# Autodesk Inventor assembly: ForeArm
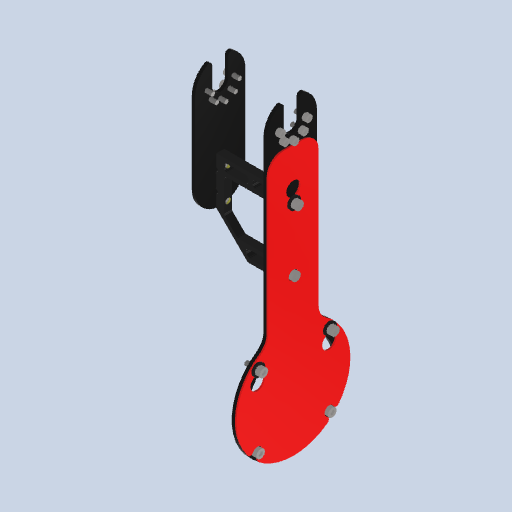
[picture p0: Inventor's stored thumbnail of the model, 512x512]
Saved by Autodesk Inventor 2022.3 (Build 263350000, 350)
## iProperties
Created: 2022-01-11
Part Number: ForeArm
Document SubType Name: Assembly
Designer: Masato Kubotera
Author: Masato Kubotera
## Documents named in this file (10)
- C:\Users\Masato\Documents\Inventor\CIT Brains\SUSTAINA-OP - mod\UpperBody\Arm\ForeArm.iam
- C:\Users\Masato\Documents\Inventor\CIT Brains\SUSTAINA-OP - mod\UpperBody\Arm\ForeArm_outside_frame.ipt
- C:\Users\Masato\Documents\Inventor\CIT Brains\SUSTAINA-OP - mod\UpperBody\Arm\ForeArm_inside_frame.ipt
- C:\Users\Masato\Documents\Inventor\CIT Brains\SUSTAINA-OP - mod\ReadyMade\Screw\UC-0306.ipt
- C:\Users\Masato\Documents\Inventor\CIT Brains\SUSTAINA-OP - mod\ReadyMade\Screw\UC-2606.ipt
- C:\Users\Masato\Documents\Inventor\CIT Brains\SUSTAINA-OP - mod\ReadyMade\InsertNut\IRU-304S.ipt
- C:\Users\Masato\Documents\Inventor\CIT Brains\SUSTAINA-OP - mod\UpperBody\Arm\ForeArm_diagonal.ipt
- C:\Users\Masato\Documents\Inventor\CIT Brains\SUSTAINA-OP - mod\UpperBody\Arm\ForeArm_outside_cloth.ipt
- C:\Users\Masato\Documents\Inventor\CIT Brains\SUSTAINA-OP - mod\ReadyMade\Bush\L3040-8110TB.ipt
- C:\Users\Masato\Documents\Inventor\CIT Brains\SUSTAINA-OP - mod\ReadyMade\Screw\UC-0308.ipt
## Components (29 placed, 9 different names)
1. ForeArm_outside_cloth:1 — 挿入:47, 挿入:48, 挿入:49
2. ForeArm_outside_frame:1 — 挿入:16, 挿入:17, 挿入:23, 挿入:24, 挿入:28, 挿入:31, 挿入:32, 挿入:33, 挿入:34, メイト:1, メイト:2, フラッシュ:1, 挿入:39, 挿入:41, 挿入:42, 挿入:43
3. ForeArm_inside_frame:1 — 挿入:25, 挿入:26, 挿入:29, 挿入:30, 挿入:35, 挿入:36, 挿入:37, 挿入:38, 挿入:40
4. ForeArm_diagonal:1 — 挿入:19, 挿入:20, 挿入:21, 挿入:22
5. L3040-8110TB:1 — 挿入:41, 挿入:47, 挿入:50
6. L3040-8110TB:2 — 挿入:42, 挿入:48, 挿入:51
7. L3040-8110TB:3 — 挿入:43, 挿入:46, 挿入:49
8. IRU-304S:1 — 挿入:19, 挿入:23
9. IRU-304S:2 — 挿入:20, 挿入:24
10. IRU-304S:3 — 挿入:21, 挿入:25
11. IRU-304S:4 — 挿入:22, 挿入:26
12. UC-2606:9 — 挿入:39
13. UC-2606:10 — 挿入:40
14. UC-2606:8 — 挿入:38
15. UC-2606:7 — 挿入:37
16. UC-2606:6 — 挿入:36
17. UC-2606:5 — 挿入:35
18. UC-2606:4 — 挿入:34
19. UC-2606:3 — 挿入:33
20. UC-2606:2 — 挿入:32
21. UC-2606:1 — 挿入:31
22. UC-0306:5 — 挿入:17
23. UC-0306:4 — 挿入:16
24. UC-0308:1 — 挿入:46
25. UC-0308:2 — 挿入:50
26. UC-0308:3 — 挿入:51
27. UC-0306:10 — 挿入:30
28. UC-0306:9 — 挿入:29
29. UC-0306:8 — 挿入:28
## Relationships (35: Insert 32, Mate 2, Flush 1)
- 挿入:16 [Insert]: ForeArm_outside_frame:1 ↔ UC-0306:4
- 挿入:17 [Insert]: ForeArm_outside_frame:1 ↔ UC-0306:5
- 挿入:19 [Insert]: ForeArm_diagonal:1 ↔ IRU-304S:1
- 挿入:20 [Insert]: ForeArm_diagonal:1 ↔ IRU-304S:2
- 挿入:21 [Insert]: ForeArm_diagonal:1 ↔ IRU-304S:3
- 挿入:22 [Insert]: ForeArm_diagonal:1 ↔ IRU-304S:4
- 挿入:23 [Insert]: ForeArm_outside_frame:1 ↔ IRU-304S:1
- 挿入:24 [Insert]: ForeArm_outside_frame:1 ↔ IRU-304S:2
- 挿入:25 [Insert]: ForeArm_inside_frame:1 ↔ IRU-304S:3
- 挿入:26 [Insert]: ForeArm_inside_frame:1 ↔ IRU-304S:4
- 挿入:28 [Insert]: ForeArm_outside_frame:1 ↔ UC-0306:8
- 挿入:29 [Insert]: ForeArm_inside_frame:1 ↔ UC-0306:9
- 挿入:30 [Insert]: ForeArm_inside_frame:1 ↔ UC-0306:10
- 挿入:31 [Insert]: ForeArm_outside_frame:1 ↔ UC-2606:1
- 挿入:32 [Insert]: ForeArm_outside_frame:1 ↔ UC-2606:2
- 挿入:33 [Insert]: ForeArm_outside_frame:1 ↔ UC-2606:3
- 挿入:34 [Insert]: ForeArm_outside_frame:1 ↔ UC-2606:4
- 挿入:35 [Insert]: ForeArm_inside_frame:1 ↔ UC-2606:5
- 挿入:36 [Insert]: ForeArm_inside_frame:1 ↔ UC-2606:6
- 挿入:37 [Insert]: ForeArm_inside_frame:1 ↔ UC-2606:7
- 挿入:38 [Insert]: ForeArm_inside_frame:1 ↔ UC-2606:8
- メイト:1 [Mate]: ForeArm_outside_frame:1
- メイト:2 [Mate]: ForeArm_outside_frame:1
- フラッシュ:1 [Flush]: ForeArm_outside_frame:1
- 挿入:39 [Insert]: ForeArm_outside_frame:1 ↔ UC-2606:9
- 挿入:40 [Insert]: ForeArm_inside_frame:1 ↔ UC-2606:10
- 挿入:41 [Insert]: ForeArm_outside_frame:1 ↔ L3040-8110TB:1
- 挿入:42 [Insert]: ForeArm_outside_frame:1 ↔ L3040-8110TB:2
- 挿入:43 [Insert]: ForeArm_outside_frame:1 ↔ L3040-8110TB:3
- 挿入:46 [Insert]: L3040-8110TB:3 ↔ UC-0308:1
- 挿入:47 [Insert]: ForeArm_outside_cloth:1 ↔ L3040-8110TB:1
- 挿入:48 [Insert]: ForeArm_outside_cloth:1 ↔ L3040-8110TB:2
- 挿入:49 [Insert]: ForeArm_outside_cloth:1 ↔ L3040-8110TB:3
- 挿入:50 [Insert]: L3040-8110TB:1 ↔ UC-0308:2
- 挿入:51 [Insert]: L3040-8110TB:2 ↔ UC-0308:3
